# Autodesk Inventor assembly: CAN_transceiver_with_pins
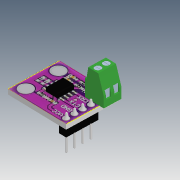
[picture p0: Inventor's stored thumbnail of the model, 180x180]
Saved by Autodesk Inventor 2020 (Build 240168000, 168)
## iProperties
Created: 2020-09-27
Part Number: CAN_transceiver_with_pins
Document SubType Name: Assembly
Designer: DELL
Author: DELL
## Documents named in this file (4)
- F:\SoftRobot\Model\FlexipodHardware-master\mechanical_model\CAN_transceiver\CAN_transceiver_with_pins.iam
- F:\SoftRobot\Model\FlexipodHardware-master\mechanical_model\CAN_transceiver\CAN_transceiver.ipt
- F:\SoftRobot\Model\FlexipodHardware-master\mechanical_model\pins.ipt
- F:\SoftRobot\Model\FlexipodHardware-master\mechanical_model\CAN_transceiver\CAN_bus_wire.ipt
## Components (6 placed, 3 different names)
1. CAN_transceiver:1 — Mate:1, Mate:2, Angle:1, Mate:3, Mate:4, Mate:5
2. CAN_bus_wire:1 — Mate:3, Mate:4, Mate:5
3. pins:1 — Mate:1, Mate:2, Angle:1
4. pins:2
5. pins:3
6. pins:4
## Component patterns: (4 elements, first: pins:1)
## Relationships (6: Mate 5, Angle 1)
- Mate:1: CAN_transceiver:1 ↔ pins:1
- Mate:2: CAN_transceiver:1 ↔ pins:1
- Angle:1 (0 deg): CAN_transceiver:1 ↔ pins:1
- Mate:3: CAN_transceiver:1 ↔ CAN_bus_wire:1
- Mate:4: CAN_transceiver:1 ↔ CAN_bus_wire:1
- Mate:5: CAN_transceiver:1 ↔ CAN_bus_wire:1
